# Autodesk Inventor assembly: Assembly
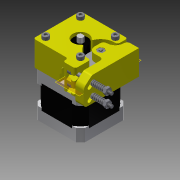
[picture p0: Inventor's stored thumbnail of the model, 180x180]
Saved by Autodesk Inventor 2013 (Build 170138000, 138)
## iProperties
Created: 2013-12-22
Part Number: Assembly
Document SubType Name: Assembly
Designer: employee
Author: employee
## Documents named in this file (12)
- C:\Users\employee\Desktop\ConceptFORGE\ConceptFORGE\FILAMENT DRIVE\INVENTOR FILES\FILAMENT DRIVE.iam
- C:\Users\employee\Desktop\ConceptFORGE\ConceptFORGE\FILAMENT DRIVE\INVENTOR FILES\_STEPPER.ipt
- C:\Users\employee\Desktop\ConceptFORGE\ConceptFORGE\FILAMENT DRIVE\INVENTOR FILES\block.ipt
- C:\Users\employee\Desktop\ConceptFORGE\ConceptFORGE\FILAMENT DRIVE\INVENTOR FILES\HOBBED PULLEY.ipt
- C:\Users\employee\Desktop\ConceptFORGE\ConceptFORGE\FILAMENT DRIVE\INVENTOR FILES\ARM.ipt
- C:\Users\employee\Desktop\ConceptFORGE\ConceptFORGE\FILAMENT DRIVE\INVENTOR FILES\BEARING INSERT.ipt
- C:\Users\employee\Desktop\ConceptFORGE\ConceptFORGE\FILAMENT DRIVE\INVENTOR FILES\_608.ipt
- C:\Users\employee\Desktop\ConceptFORGE\ConceptFORGE\FILAMENT DRIVE\INVENTOR FILES\SPRING.ipt
- C:\Users\employee\Desktop\ConceptFORGE\ConceptFORGE\FILAMENT DRIVE\INVENTOR FILES\M3x35.ipt
- C:\Users\employee\Desktop\ConceptFORGE\ConceptFORGE\FILAMENT DRIVE\INVENTOR FILES\M3 NUT.ipt
- C:\Users\employee\Desktop\ConceptFORGE\ConceptFORGE\FILAMENT DRIVE\INVENTOR FILES\M3x20.ipt
- C:\Users\employee\Desktop\ConceptFORGE\ConceptFORGE\FILAMENT DRIVE\INVENTOR FILES\M3x25.ipt
## Components (18 placed, 11 different names)
1. _STEPPER:1 — Insert:1, Angle:1, Mate:1, Flush:1, Insert:14
2. block:1 — Insert:1, Angle:1, Mate:2, Insert:4, Insert:5, Insert:10, Insert:11, Insert:12, Insert:13, Angle:3
3. HOBBED PULLEY:1 — Mate:1, Mate:2
4. ARM:1 — Flush:1, Insert:2, Mate:3, Mate:4, Tangent:1, Tangent:2, Insert:8, Angle:2, Insert:9, Insert:14, Angle:3
5. BEARING INSERT:1 — Insert:2, Insert:3
6. _608:1 — Insert:3
7. SPRING:1 — Mate:3, Tangent:2
8. SPRING:2 — Mate:4, Tangent:1
9. M3x35:1 — Insert:4, Insert:6
10. M3x35:2 — Insert:5, Insert:7
11. M3 NUT:1 — Insert:7
12. M3 NUT:2 — Insert:6
13. M3 NUT:3 — Insert:8, Angle:2
14. M3x20:1 — Insert:9
15. M3x25:1 — Insert:10
16. M3x25:2 — Insert:11
17. M3x25:3 — Insert:13
18. M3x25:4 — Insert:12
## Relationships (24: Insert 14, Mate 4, Angle 3, Tangent 2, Flush 1)
- Insert:1: _STEPPER:1 ↔ block:1
- Angle:1 (0 deg): _STEPPER:1 ↔ block:1
- Mate:1: _STEPPER:1 ↔ HOBBED PULLEY:1
- Mate:2 (-11.27 mm): block:1 ↔ HOBBED PULLEY:1
- Flush:1: _STEPPER:1 ↔ ARM:1
- Insert:2 (0.1 mm): ARM:1 ↔ BEARING INSERT:1
- Insert:3: BEARING INSERT:1 ↔ _608:1
- Mate:3: ARM:1 ↔ SPRING:1
- Mate:4: ARM:1 ↔ SPRING:2
- Tangent:1: ARM:1 ↔ SPRING:2
- Tangent:2: ARM:1 ↔ SPRING:1
- Insert:4: block:1 ↔ M3x35:1
- Insert:5: block:1 ↔ M3x35:2
- Insert:6 (3.3 mm): M3x35:1 ↔ M3 NUT:2
- Insert:7 (3.3 mm): M3x35:2 ↔ M3 NUT:1
- Insert:8: ARM:1 ↔ M3 NUT:3
- Angle:2 (0 deg): ARM:1 ↔ M3 NUT:3
- Insert:9: ARM:1 ↔ M3x20:1
- Insert:10: block:1 ↔ M3x25:1
- Insert:11: block:1 ↔ M3x25:2
- Insert:12: block:1 ↔ M3x25:4
- Insert:13: block:1 ↔ M3x25:3
- Insert:14: _STEPPER:1 ↔ ARM:1
- Angle:3 (0 deg): block:1 ↔ ARM:1
